# Autodesk Inventor assembly: WalkCat
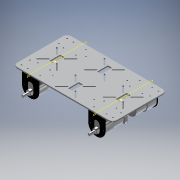
[picture p0: Inventor's stored thumbnail of the model, 180x180]
Saved by Autodesk Inventor 2018 (Build 220112000, 112)
## iProperties
Created: 2021-04-30
Part Number: WalkCat
Document SubType Name: Assembly
Designer: dangl
Author: dangl
## Documents named in this file (4)
- C:\Users\dangl\Desktop\Ender3 Pro\My Prints\WalkCat\WalkCat.iam
- C:\Users\dangl\Desktop\Ender3 Pro\My Prints\WalkCat\Base.ipt
- C:\Users\dangl\Desktop\Ender3 Pro\My Prints\WalkCat\MotorMount.ipt
- C:\Users\dangl\Desktop\Ender3 Pro\My Prints\WalkCat\Motor.ipt
## Components (9 placed, 3 different names)
1. Base:1 — Mate:1, Mate:2, Mate:3, Mate:4, Mate:5, Mate:6, Mate:7, Mate:8, Mate:9, Mate:10, Mate:11, Mate:12
2. MotorMount:1 — Mate:1, Mate:5, Mate:6, Mate:13, Mate:14, Mate:15
3. MotorMount:2 — Mate:2, Mate:7, Mate:8, Mate:16, Mate:21, Mate:22
4. MotorMount:3 — Mate:3, Mate:11, Mate:12, Mate:18, Mate:20, Mate:23
5. MotorMount:4 — Mate:4, Mate:9, Mate:10, Mate:17, Mate:19, Mate:24
6. Motor:1 — Mate:13, Mate:14, Mate:15
7. Motor:2 — Mate:16, Mate:21, Mate:22
8. Motor:3 — Mate:17, Mate:19, Mate:24
9. Motor:4 — Mate:18, Mate:20, Mate:23
## Relationships (24: Mate 24)
- Mate:1: Base:1 ↔ MotorMount:1
- Mate:2: Base:1 ↔ MotorMount:2
- Mate:3: Base:1 ↔ MotorMount:3
- Mate:4: Base:1 ↔ MotorMount:4
- Mate:5: Base:1 ↔ MotorMount:1
- Mate:6: Base:1 ↔ MotorMount:1
- Mate:7: Base:1 ↔ MotorMount:2
- Mate:8: Base:1 ↔ MotorMount:2
- Mate:9: Base:1 ↔ MotorMount:4
- Mate:10: Base:1 ↔ MotorMount:4
- Mate:11: Base:1 ↔ MotorMount:3
- Mate:12: Base:1 ↔ MotorMount:3
- Mate:13: MotorMount:1 ↔ Motor:1
- Mate:14: MotorMount:1 ↔ Motor:1
- Mate:15: MotorMount:1 ↔ Motor:1
- Mate:16: MotorMount:2 ↔ Motor:2
- Mate:17: MotorMount:4 ↔ Motor:3
- Mate:18: MotorMount:3 ↔ Motor:4
- Mate:19: MotorMount:4 ↔ Motor:3
- Mate:20: MotorMount:3 ↔ Motor:4
- Mate:21: MotorMount:2 ↔ Motor:2
- Mate:22: MotorMount:2 ↔ Motor:2
- Mate:23: MotorMount:3 ↔ Motor:4
- Mate:24: MotorMount:4 ↔ Motor:3
